# Autodesk Inventor assembly: Assembly1
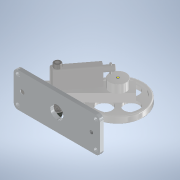
[picture p0: Inventor's stored thumbnail of the model, 180x180]
Saved by Autodesk Inventor 2022.2 (Build 262287010, 287A)
## iProperties
Created: 2022-05-04
Part Number: Assembly1
Document SubType Name: Assembly
Designer: Korch
Author: Korch
## Documents named in this file (16)
- C:\Users\Usuario\Desktop\Faculdade\modelagem_3D\motor_cilindro_unico\Assembly1.iam
- C:\Users\Usuario\Desktop\Faculdade\modelagem_3D\motor_cilindro_unico\base_plate.ipt
- C:\Users\Usuario\Desktop\Faculdade\modelagem_3D\motor_cilindro_unico\main_frame.ipt
- C:\Users\Usuario\Documents\Inventor\Content Center Files\R2022\en-US\ISO 4762(2)\ISO 4762 - M6 x 12ISO.ipt
- C:\Users\Usuario\Desktop\Faculdade\modelagem_3D\motor_cilindro_unico\Air_hose_coupling.ipt
- C:\Users\Usuario\Desktop\Faculdade\modelagem_3D\motor_cilindro_unico\cilinder.ipt
- C:\Users\Usuario\Documents\Inventor\Content Center Files\R2022\en-US\ISO 4762(2)\ISO 4762 - M6 x 60ISO.ipt
- C:\Users\Usuario\Desktop\Faculdade\modelagem_3D\motor_cilindro_unico\mola.ipt
- C:\Users\Usuario\Documents\Inventor\Content Center Files\R2022\en-US\BS EN 24034\ISO 4034 - M6BS EN.ipt
- C:\Users\Usuario\Documents\Inventor\Content Center Files\R2022\en-US\AS 1237 (2.1)\AS 1237 - 6.ipt
- C:\Users\Usuario\Desktop\Faculdade\modelagem_3D\motor_cilindro_unico\crank_wheel.ipt
- C:\Users\Usuario\Desktop\Faculdade\modelagem_3D\motor_cilindro_unico\fly_wheel.ipt
- C:\Users\Usuario\Desktop\Faculdade\modelagem_3D\motor_cilindro_unico\crank_shaft.ipt
- C:\Users\Usuario\Desktop\Faculdade\modelagem_3D\motor_cilindro_unico\piston.ipt
- C:\Users\Usuario\Desktop\Faculdade\modelagem_3D\motor_cilindro_unico\crank_pin.ipt
- C:\Users\Usuario\Documents\Inventor\Content Center Files\R2022\en-US\ISO 4027\ISO 4027 - M2,5 x 6 - ISO.ipt
## Components (15 placed, 15 different names)
1. base_plate:1 — Rigid:1
2. main_frame:1 — Rigid:1, Mate:1, Mate:2, Rotational:1, Rotational:2, Rotational:4
3. ISO 4762 M6 x 12:1 — Mate:1, Mate:2
4. Air_hose_coupling:1 — Rotational:1
5. cilinder:1 — Rotational:2, Mate:3, Mate:4, Cylindrical:1
6. ISO 4762 M6 x 60:1 — Mate:3, Mate:4, Mate:5, Rigid:2
7. mola:1 — Mate:5
8. BS EN 24034 - Metric M6:1 — Rotational:3
9. AS 1237 (2.1) 6:1 — Rigid:2, Rotational:3
10. crank_wheel:1 — Rotational:4, Rigid:3, Rotational:6
11. fly_wheel:1 — Rigid:4, Rigid:5
12. crank_shaft:1 — Rigid:3, Rigid:5
13. piston:1 — Cylindrical:1, Mate:6
14. crank_pin:1 — Rotational:6, Mate:6
15. ISO 4027 M2,5 x 6:1 — Rigid:4
## Relationships (18: Mate 6, WeldJoint 5, RevoluteJoint 5, Flush 1, CylindricalJoint 1)
- Rigid:1 [WeldJoint]: base_plate:1 ↔ main_frame:1
- Mate:1: main_frame:1 ↔ ISO 4762 M6 x 12:1
- Mate:2: main_frame:1 ↔ ISO 4762 M6 x 12:1
- Rotational:1 [RevoluteJoint]: main_frame:1 ↔ Air_hose_coupling:1
- Rotational:2 [RevoluteJoint]: main_frame:1 ↔ cilinder:1
- Mate:3: cilinder:1 ↔ ISO 4762 M6 x 60:1
- Mate:4: cilinder:1 ↔ ISO 4762 M6 x 60:1
- Flush:1 (-20 mm)
- Mate:5: ISO 4762 M6 x 60:1 ↔ mola:1
- Rigid:2 [WeldJoint] (-4.4 mm): ISO 4762 M6 x 60:1 ↔ AS 1237 (2.1) 6:1
- Rotational:3 [RevoluteJoint] (-0.1 mm): BS EN 24034 - Metric M6:1 ↔ AS 1237 (2.1) 6:1
- Rotational:4 [RevoluteJoint]: main_frame:1 ↔ crank_wheel:1
- Rigid:3 [WeldJoint]: crank_wheel:1 ↔ crank_shaft:1
- Cylindrical:1: cilinder:1 ↔ piston:1
- Rotational:6 [RevoluteJoint]: crank_wheel:1 ↔ crank_pin:1
- Mate:6: piston:1 ↔ crank_pin:1
- Rigid:4 [WeldJoint]: fly_wheel:1 ↔ ISO 4027 M2,5 x 6:1
- Rigid:5 [WeldJoint]: fly_wheel:1 ↔ crank_shaft:1
